# Autodesk Inventor assembly: GE-17088_ASM_44_ASM
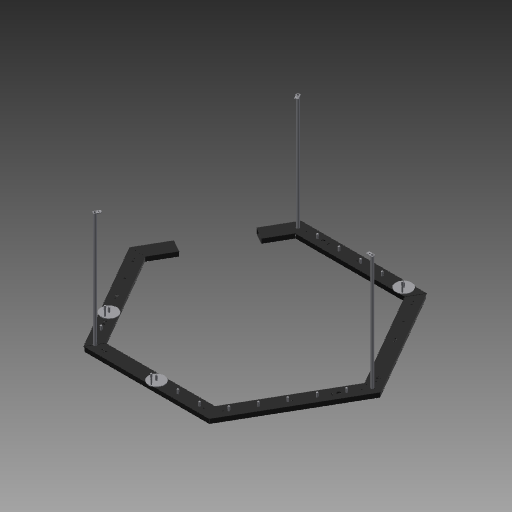
[picture p0: Inventor's stored thumbnail of the model, 512x512]
Saved by Autodesk Inventor 2017.1 (Build 211199000, 199)
## iProperties
Created: 2016-12-16
Part Number: GE-17088_ASM_44_ASM
Document SubType Name: Assembly
Designer: PhillipD
Author: PhillipD
Revision Number: 1LAST_VERSION
## Documents named in this file (15)
- D:\FIRST\FIRST KOP 2017\FRC 2017 Field\Parts\GE-17088_ASM_44_ASM.iam
- D:\FIRST\FIRST KOP 2017\FRC 2017 Field\Parts\GE-17086_27.ipt
- D:\FIRST\FIRST KOP 2017\FRC 2017 Field\Parts\GE-17222_5.ipt
- D:\FIRST\FIRST KOP 2017\FRC 2017 Field\Parts\GE-17223_2.ipt
- D:\FIRST\FIRST KOP 2017\FRC 2017 Field\Parts\GE-17087_11.ipt
- D:\FIRST\FIRST KOP 2017\FRC 2017 Field\Parts\GE-17089_ASM_8_ASM.iam
- D:\FIRST\FIRST KOP 2017\FRC 2017 Field\Parts\GE-17220_3.ipt
- D:\FIRST\FIRST KOP 2017\FRC 2017 Field\Parts\GE-17090_19.ipt
- D:\FIRST\FIRST KOP 2017\FRC 2017 Field\Parts\GE-17091_38.ipt
- D:\FIRST\FIRST KOP 2017\FRC 2017 Field\Parts\GE-17094_8.ipt
- D:\FIRST\FIRST KOP 2017\FRC 2017 Field\Parts\GE-17095_7.ipt
- D:\FIRST\FIRST KOP 2017\FRC 2017 Field\Parts\GE-17096_1.ipt
- D:\FIRST\FIRST KOP 2017\FRC 2017 Field\Parts\GE-17097_9.ipt
- D:\FIRST\FIRST KOP 2017\FRC 2017 Field\Parts\GE-17224_3.ipt
- D:\FIRST\FIRST KOP 2017\FRC 2017 Field\Parts\GE-17225_2.ipt
## Components (44 placed, 44 different names)
1. GE-17086_27_1230 — Insert:3, Insert:4
2. GE-17086_27_1231 — Insert:1
3. GE-17086_27_1232 — Insert:2, Insert:20
4. GE-17086_27_1233 — Insert:5, Insert:9
5. GE-17086_27_1234 — Insert:6
6. GE-17222_5_1235
7. GE-17223_2_1236
8. GE-17087_11_1237
9. GE-17087_11_1238
10. GE-17087_11_1239
11. GE-17087_11_1240
12. GE-17087_11_1241
13. GE-17087_11_1242
14. GE-17087_11_1243
15. GE-17087_11_1244
16. GE-17087_11_1245
17. GE-17087_11_1246 — Insert:20
18. GE-17087_11_1247
19. GE-17087_11_1248
20. GE-17089_ASM_8_ASM_1252 [sub-assembly] — Insert:3, Insert:4
21. GE-17089_ASM_8_ASM_1253 [sub-assembly] — Insert:1, Insert:2
22. GE-17089_ASM_8_ASM_1254 [sub-assembly] — Insert:5, Insert:6
23. GE-17220_3_1255 — Insert:15
24. GE-17220_3_1256 — Insert:9, Insert:10
25. GE-17220_3_1257 — Insert:13
26. GE-17090_19_1258
27. GE-17090_19_1259
28. GE-17090_19_1260
29. GE-17091_38_1261
30. GE-17091_38_1262
31. GE-17094_8_1263 — Insert:8, Insert:10, Insert:11
32. GE-17094_8_1264 — Insert:13, Insert:14, Insert:19
33. GE-17094_8_1265 — Insert:15, Insert:16, Insert:18
34. GE-17095_7_1266 — Insert:7, Insert:8
35. GE-17095_7_1267 — Insert:12, Insert:14
36. GE-17095_7_1268 — Insert:17, Insert:18
37. GE-17096_1_1269 — Insert:7
38. GE-17096_1_1270 — Insert:12
39. GE-17096_1_1271 — Insert:17
40. GE-17097_9_1272 — Insert:11
41. GE-17097_9_1273 — Insert:19
42. GE-17097_9_1274 — Insert:16
43. GE-17224_3_1275
44. GE-17225_2_1276
## Relationships (20: Insert 20)
- Insert:1: GE-17086_27_1231 ↔ GE-17089_ASM_8_ASM_1253
- Insert:2: GE-17086_27_1232 ↔ GE-17089_ASM_8_ASM_1253
- Insert:3: GE-17086_27_1230 ↔ GE-17089_ASM_8_ASM_1252
- Insert:4: GE-17086_27_1230 ↔ GE-17089_ASM_8_ASM_1252
- Insert:5: GE-17086_27_1233 ↔ GE-17089_ASM_8_ASM_1254
- Insert:6: GE-17086_27_1234 ↔ GE-17089_ASM_8_ASM_1254
- Insert:7: GE-17095_7_1266 ↔ GE-17096_1_1269
- Insert:8: GE-17094_8_1263 ↔ GE-17095_7_1266
- Insert:9: GE-17086_27_1233 ↔ GE-17220_3_1256
- Insert:10: GE-17220_3_1256 ↔ GE-17094_8_1263
- Insert:11: GE-17094_8_1263 ↔ GE-17097_9_1272
- Insert:12: GE-17095_7_1267 ↔ GE-17096_1_1270
- Insert:13: GE-17220_3_1257 ↔ GE-17094_8_1264
- Insert:14: GE-17094_8_1264 ↔ GE-17095_7_1267
- Insert:15: GE-17220_3_1255 ↔ GE-17094_8_1265
- Insert:16: GE-17094_8_1265 ↔ GE-17097_9_1274
- Insert:17: GE-17095_7_1268 ↔ GE-17096_1_1271
- Insert:18: GE-17094_8_1265 ↔ GE-17095_7_1268
- Insert:19: GE-17094_8_1264 ↔ GE-17097_9_1273
- Insert:20: GE-17086_27_1232 ↔ GE-17087_11_1246
